# Autodesk Inventor assembly: Cartridge assembly
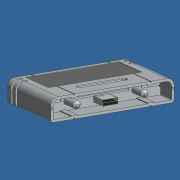
[picture p0: Inventor's stored thumbnail of the model, 180x180]
Saved by Autodesk Inventor 2021 (Build 250183000, 183)
## iProperties
Created: 2022-08-19
Part Number: Cartridge assembly
Document SubType Name: Assembly
Designer: Usuario
Author: Usuario
Revision Number: 01
## Documents named in this file (5)
- J:\Codigo\C++\Vircon32\PhysicalElements\Cartridges\Cartridge assembly.iam
- J:\Codigo\C++\Vircon32\PhysicalElements\Cartridges\Cartridge back half.ipt
- J:\Codigo\C++\Vircon32\PhysicalElements\Cartridges\Reference USB stick with hole.ipt
- J:\Codigo\C++\Vircon32\PhysicalElements\Cartridges\Self tappping screw DIN 7981-C Ø2.9x9.5.ipt
- J:\Codigo\C++\Vircon32\PhysicalElements\Cartridges\Cartridge front half.ipt
## Components (5 placed, 4 different names)
1. Cartridge back half:1 — Insertar:1, Insertar:2, Insertar:3
2. Cartridge front half:1
3. Reference USB stick with hole:1 — Insertar:1, Coincidencia:1
4. Self tappping screw DIN 7981-C Ø2.9x9.5:1 — Insertar:2
5. Self tappping screw DIN 7981-C Ø2.9x9.5:2 — Insertar:3
## Relationships (4: Insert 3, Mate 1)
- Insertar:1 (0.1 mm): Cartridge back half:1 ↔ Reference USB stick with hole:1
- Coincidencia:1 [Mate]: Reference USB stick with hole:1
- Insertar:2: Cartridge back half:1 ↔ Self tappping screw DIN 7981-C Ø2.9x9.5:1
- Insertar:3: Cartridge back half:1 ↔ Self tappping screw DIN 7981-C Ø2.9x9.5:2
